# Autodesk Inventor assembly: robot_frame
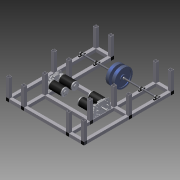
[picture p0: Inventor's stored thumbnail of the model, 180x180]
Saved by Autodesk Inventor 2011 (Build 150239000, 239)
## iProperties
Created: 2013-01-17
Part Number: robot_frame
Document SubType Name: Assembly
Designer: Christopher
Author: Christopher
## Documents named in this file (3)
- F:\Users\Christopher\Documents\GitHub\2013CAD\2013 robot\forklift\robot parts\robot_frame.iam
- F:\Users\Christopher\Documents\GitHub\2013CAD\2013 robot\forklift\robot parts\robot_frame_layer1.iam
- F:\Users\Christopher\Documents\GitHub\2013CAD\2013 robot\forklift\robot parts\1tube_6_midlayer.ipt
## Components (15 placed, 2 different names)
1. robot_frame_layer1:1 [sub-assembly] — Mate:1, Flush:1, Mate:2, Mate:3, Mate:4, Mate:5, Mate:6, Flush:2, Flush:3, Mate:7, Flush:4, Flush:5, Mate:8, Mate:9, Mate:10, Mate:11, Mate:12, Mate:13, Mate:14, Mate:15, Mate:16, Mate:17, Mate:18, Mate:19, Mate:20, Mate:21, Mate:22, Mate:23, Mate:24, Mate:25, Mate:26, Mate:27, Mate:28, Mate:29, Mate:30, Mate:31, Mate:32, Mate:33, Mate:34, Mate:35, Mate:36, Mate:37
2. 1tube_6_midlayer:1 — Mate:3, Mate:4, Mate:5
3. 1tube_6_midlayer:2 — Mate:8, Mate:9, Mate:10
4. 1tube_6_midlayer:3 — Mate:17, Mate:18, Mate:19
5. 1tube_6_midlayer:4 — Mate:14, Mate:15, Mate:16
6. 1tube_6_midlayer:5 — Mate:7, Flush:4, Flush:5
7. 1tube_6_midlayer:6 — Mate:6, Flush:2, Flush:3
8. 1tube_6_midlayer:7 — Mate:1, Flush:1, Mate:2
9. 1tube_6_midlayer:8 — Mate:11, Mate:12, Mate:13
10. 1tube_6_midlayer:9 — Mate:20, Mate:21, Mate:22
11. 1tube_6_midlayer:10 — Mate:23, Mate:24, Mate:25
12. 1tube_6_midlayer:11 — Mate:26, Mate:27, Mate:28
13. 1tube_6_midlayer:12 — Mate:29, Mate:30, Mate:31
14. 1tube_6_midlayer:13 — Mate:32, Mate:33, Mate:34
15. 1tube_6_midlayer:14 — Mate:35, Mate:36, Mate:37
## Relationships (42: Mate 37, Flush 5)
- Mate:1: robot_frame_layer1:1 ↔ 1tube_6_midlayer:7
- Flush:1: robot_frame_layer1:1 ↔ 1tube_6_midlayer:7
- Mate:2: robot_frame_layer1:1 ↔ 1tube_6_midlayer:7
- Mate:3: robot_frame_layer1:1 ↔ 1tube_6_midlayer:1
- Mate:4: robot_frame_layer1:1 ↔ 1tube_6_midlayer:1
- Mate:5: robot_frame_layer1:1 ↔ 1tube_6_midlayer:1
- Mate:6: robot_frame_layer1:1 ↔ 1tube_6_midlayer:6
- Flush:2: robot_frame_layer1:1 ↔ 1tube_6_midlayer:6
- Flush:3: robot_frame_layer1:1 ↔ 1tube_6_midlayer:6
- Mate:7: robot_frame_layer1:1 ↔ 1tube_6_midlayer:5
- Flush:4: robot_frame_layer1:1 ↔ 1tube_6_midlayer:5
- Flush:5: robot_frame_layer1:1 ↔ 1tube_6_midlayer:5
- Mate:8: robot_frame_layer1:1 ↔ 1tube_6_midlayer:2
- Mate:9: robot_frame_layer1:1 ↔ 1tube_6_midlayer:2
- Mate:10: robot_frame_layer1:1 ↔ 1tube_6_midlayer:2
- Mate:11: robot_frame_layer1:1 ↔ 1tube_6_midlayer:8
- Mate:12: robot_frame_layer1:1 ↔ 1tube_6_midlayer:8
- Mate:13: robot_frame_layer1:1 ↔ 1tube_6_midlayer:8
- Mate:14: robot_frame_layer1:1 ↔ 1tube_6_midlayer:4
- Mate:15: robot_frame_layer1:1 ↔ 1tube_6_midlayer:4
- Mate:16: robot_frame_layer1:1 ↔ 1tube_6_midlayer:4
- Mate:17: robot_frame_layer1:1 ↔ 1tube_6_midlayer:3
- Mate:18: robot_frame_layer1:1 ↔ 1tube_6_midlayer:3
- Mate:19: robot_frame_layer1:1 ↔ 1tube_6_midlayer:3
- Mate:20: robot_frame_layer1:1 ↔ 1tube_6_midlayer:9
- Mate:21: robot_frame_layer1:1 ↔ 1tube_6_midlayer:9
- Mate:22: robot_frame_layer1:1 ↔ 1tube_6_midlayer:9
- Mate:23: robot_frame_layer1:1 ↔ 1tube_6_midlayer:10
- Mate:24: robot_frame_layer1:1 ↔ 1tube_6_midlayer:10
- Mate:25: robot_frame_layer1:1 ↔ 1tube_6_midlayer:10
- Mate:26: robot_frame_layer1:1 ↔ 1tube_6_midlayer:11
- Mate:27: robot_frame_layer1:1 ↔ 1tube_6_midlayer:11
- Mate:28: robot_frame_layer1:1 ↔ 1tube_6_midlayer:11
- Mate:29: robot_frame_layer1:1 ↔ 1tube_6_midlayer:12
- Mate:30: robot_frame_layer1:1 ↔ 1tube_6_midlayer:12
- Mate:31: robot_frame_layer1:1 ↔ 1tube_6_midlayer:12
- Mate:32: robot_frame_layer1:1 ↔ 1tube_6_midlayer:13
- Mate:33: robot_frame_layer1:1 ↔ 1tube_6_midlayer:13
- Mate:34: robot_frame_layer1:1 ↔ 1tube_6_midlayer:13
- Mate:35: robot_frame_layer1:1 ↔ 1tube_6_midlayer:14
- Mate:36: robot_frame_layer1:1 ↔ 1tube_6_midlayer:14
- Mate:37: robot_frame_layer1:1 ↔ 1tube_6_midlayer:14
